# Autodesk Inventor assembly: PinionGearV2
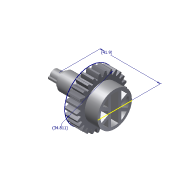
[picture p0: Inventor's stored thumbnail of the model, 180x180]
Saved by Autodesk Inventor 2012 (Build 160160000, 160)
## iProperties
Created: 2017-01-26
Part Number: PinionGearV2
Document SubType Name: Assembly
Designer: omaro
Mass: 28.428 g
Surface Area: 26.386 cm^2
Volume: 3.6214 cm^3
Density: 7.85 g/cm^3
Author: omaro
## Documents named in this file (3)
- C:\Users\omaro\Desktop\Gate_Model\Gate Motor Gears\_V2\PinionGearV2.iam
- C:\Users\omaro\Desktop\Gate_Model\Gate Motor Gears\_V2\DrivingShaft.ipt
- C:\Users\omaro\Desktop\Gate_Model\Gate Motor Gears\_V2\PinionGear\Design Accelerator\Spur Gears1.iam
## Components (2 placed, 2 different names)
1. DrivingShaft:1 — Mate:1, Flush:1
2. Spur Gears:1 [sub-assembly] — Mate:1, Flush:1
## Relationships (2: Mate 1, Flush 1)
- Mate:1: DrivingShaft:1 ↔ Spur Gears:1
- Flush:1 (8.9 mm): DrivingShaft:1 ↔ Spur Gears:1
